# Autodesk Inventor assembly: Pan_Tilt
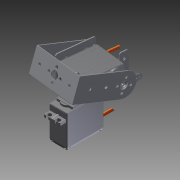
[picture p0: Inventor's stored thumbnail of the model, 180x180]
Saved by Autodesk Inventor 2015 (Build 190159000, 159)
## iProperties
Created: 2015-03-10
Part Number: Pan_Tilt
Document SubType Name: Assembly
Designer: ChristopherEvan
Author: ChristopherEvan
## Documents named in this file (4)
- C:\Users\ChristopherEvan\Documents\Inventor\MAKE\Pan_Tilt\Pan_Tilt.iam
- C:\Users\ChristopherEvan\Documents\Inventor\MAKE\Pan_Tilt\Servo\TOWER PRO MG-995, ANALOG SERVO.iam
- C:\Users\ChristopherEvan\Documents\Inventor\MAKE\Pan_Tilt\Bracket.ipt
- C:\Users\ChristopherEvan\Documents\Inventor\MAKE\Pan_Tilt\C_Bracket.ipt
## Components (4 placed, 3 different names)
1. TOWER PRO MG-995, ANALOG SERVO:1 [sub-assembly] — Mate:1, Mate:2
2. Bracket:1 — Mate:1, Mate:2, Mate:3, Mate:4, Angle:1
3. TOWER PRO MG-995, ANALOG SERVO:2 [sub-assembly] — Mate:3, Mate:4, Angle:1, Mate:5, Mate:6
4. C_Bracket:1 — Mate:5, Mate:6
## Relationships (7: Mate 6, Angle 1)
- Mate:1: TOWER PRO MG-995, ANALOG SERVO:1 ↔ Bracket:1
- Mate:2: TOWER PRO MG-995, ANALOG SERVO:1 ↔ Bracket:1
- Mate:3: Bracket:1 ↔ TOWER PRO MG-995, ANALOG SERVO:2
- Mate:4: Bracket:1 ↔ TOWER PRO MG-995, ANALOG SERVO:2
- Angle:1 (0 deg): Bracket:1 ↔ TOWER PRO MG-995, ANALOG SERVO:2
- Mate:5: TOWER PRO MG-995, ANALOG SERVO:2 ↔ C_Bracket:1
- Mate:6: TOWER PRO MG-995, ANALOG SERVO:2 ↔ C_Bracket:1
